# Autodesk Inventor assembly: 810004_X0X
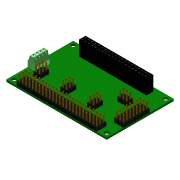
[picture p0: Inventor's stored thumbnail of the model, 180x180]
Saved by Autodesk Inventor 2015 (Build 190159000, 159)
## iProperties
Created: 2014-08-28
Part Number: 810004_X0X
Document SubType Name: Assembly
Designer: david
Author: david
## Documents named in this file (3)
- C:\SharedDrive\Dropbox\FAST Robotics\Products\818004_Power Shield\MECH\810004_Power Shield\810004A\810004A_X0X.iam
- C:\SharedDrive\Dropbox\FAST Robotics\Products\818004_Power Shield\MECH\810004_Power Shield\810004A\810004A_XXX.iam
- C:\SharedDrive\Dropbox\FAST Robotics\Library\784001_CONN HEADER .1in SINGLE STR 40POS\CONN HEADER .1in SINGLE STR 40POS.ipt
## Components (97 placed, 2 different names)
1. 810004A_XXX:1 [sub-assembly] — Flush:1, Flush:2, Flush:3, Mate:1, Mate:2, Mate:3, Mate:4, Flush:4, Flush:5, Flush:6, Flush:7, Flush:8, Flush:10, Flush:11
2. CONN HEADER .1in SINGLE STR 40POS:1
3. CONN HEADER .1in SINGLE STR 40POS:2
4. CONN HEADER .1in SINGLE STR 40POS:3 — Mate:1, Flush:4, Flush:8
5. CONN HEADER .1in SINGLE STR 40POS:4
6. CONN HEADER .1in SINGLE STR 40POS:5
7. CONN HEADER .1in SINGLE STR 40POS:6
8. CONN HEADER .1in SINGLE STR 40POS:7
9. CONN HEADER .1in SINGLE STR 40POS:8
10. CONN HEADER .1in SINGLE STR 40POS:9
11. CONN HEADER .1in SINGLE STR 40POS:10
12. CONN HEADER .1in SINGLE STR 40POS:11
13. CONN HEADER .1in SINGLE STR 40POS:12
14. CONN HEADER .1in SINGLE STR 40POS:13
15. CONN HEADER .1in SINGLE STR 40POS:14
16. CONN HEADER .1in SINGLE STR 40POS:15
17. CONN HEADER .1in SINGLE STR 40POS:16
18. CONN HEADER .1in SINGLE STR 40POS:17
19. CONN HEADER .1in SINGLE STR 40POS:18
20. CONN HEADER .1in SINGLE STR 40POS:19
21. CONN HEADER .1in SINGLE STR 40POS:20
22. CONN HEADER .1in SINGLE STR 40POS:21
23. CONN HEADER .1in SINGLE STR 40POS:22
24. CONN HEADER .1in SINGLE STR 40POS:23
25. CONN HEADER .1in SINGLE STR 40POS:24 — Mate:5
26. CONN HEADER .1in SINGLE STR 40POS:25
27. CONN HEADER .1in SINGLE STR 40POS:28
28. CONN HEADER .1in SINGLE STR 40POS:29
29. CONN HEADER .1in SINGLE STR 40POS:30
30. CONN HEADER .1in SINGLE STR 40POS:31
31. CONN HEADER .1in SINGLE STR 40POS:32
32. CONN HEADER .1in SINGLE STR 40POS:33
33. CONN HEADER .1in SINGLE STR 40POS:34
34. CONN HEADER .1in SINGLE STR 40POS:35
35. CONN HEADER .1in SINGLE STR 40POS:36
36. CONN HEADER .1in SINGLE STR 40POS:37
37. CONN HEADER .1in SINGLE STR 40POS:38
38. CONN HEADER .1in SINGLE STR 40POS:39
39. CONN HEADER .1in SINGLE STR 40POS:40
40. CONN HEADER .1in SINGLE STR 40POS:41
41. CONN HEADER .1in SINGLE STR 40POS:42
42. CONN HEADER .1in SINGLE STR 40POS:43 — Mate:5
43. CONN HEADER .1in SINGLE STR 40POS:44
44. CONN HEADER .1in SINGLE STR 40POS:45
45. CONN HEADER .1in SINGLE STR 40POS:46
46. CONN HEADER .1in SINGLE STR 40POS:47 — Mate:2
47. CONN HEADER .1in SINGLE STR 40POS:48
48. CONN HEADER .1in SINGLE STR 40POS:49
49. CONN HEADER .1in SINGLE STR 40POS:50 — Flush:5
50. CONN HEADER .1in SINGLE STR 40POS:27
51. CONN HEADER .1in SINGLE STR 40POS:51
52. CONN HEADER .1in SINGLE STR 40POS:52
53. CONN HEADER .1in SINGLE STR 40POS:53
54. CONN HEADER .1in SINGLE STR 40POS:54
55. CONN HEADER .1in SINGLE STR 40POS:55
56. CONN HEADER .1in SINGLE STR 40POS:56
57. CONN HEADER .1in SINGLE STR 40POS:57 — Mate:4
58. CONN HEADER .1in SINGLE STR 40POS:58
59. CONN HEADER .1in SINGLE STR 40POS:59
60. CONN HEADER .1in SINGLE STR 40POS:60
61. CONN HEADER .1in SINGLE STR 40POS:61
62. CONN HEADER .1in SINGLE STR 40POS:62
63. CONN HEADER .1in SINGLE STR 40POS:63
64. CONN HEADER .1in SINGLE STR 40POS:64
65. CONN HEADER .1in SINGLE STR 40POS:65 — Flush:10
66. CONN HEADER .1in SINGLE STR 40POS:66
67. CONN HEADER .1in SINGLE STR 40POS:67
68. CONN HEADER .1in SINGLE STR 40POS:68
69. CONN HEADER .1in SINGLE STR 40POS:69
70. CONN HEADER .1in SINGLE STR 40POS:70
71. CONN HEADER .1in SINGLE STR 40POS:71
72. CONN HEADER .1in SINGLE STR 40POS:72 — Flush:7
73. CONN HEADER .1in SINGLE STR 40POS:73
74. CONN HEADER .1in SINGLE STR 40POS:26
75. CONN HEADER .1in SINGLE STR 40POS:74
76. CONN HEADER .1in SINGLE STR 40POS:75
77. CONN HEADER .1in SINGLE STR 40POS:76
78. CONN HEADER .1in SINGLE STR 40POS:77
79. CONN HEADER .1in SINGLE STR 40POS:78
80. CONN HEADER .1in SINGLE STR 40POS:79
81. CONN HEADER .1in SINGLE STR 40POS:80
82. CONN HEADER .1in SINGLE STR 40POS:81
83. CONN HEADER .1in SINGLE STR 40POS:82
84. CONN HEADER .1in SINGLE STR 40POS:83
85. CONN HEADER .1in SINGLE STR 40POS:84
86. CONN HEADER .1in SINGLE STR 40POS:85
87. CONN HEADER .1in SINGLE STR 40POS:86
88. CONN HEADER .1in SINGLE STR 40POS:87
89. CONN HEADER .1in SINGLE STR 40POS:88
90. CONN HEADER .1in SINGLE STR 40POS:89 — Flush:11
91. CONN HEADER .1in SINGLE STR 40POS:90
92. CONN HEADER .1in SINGLE STR 40POS:91
93. CONN HEADER .1in SINGLE STR 40POS:92
94. CONN HEADER .1in SINGLE STR 40POS:93
95. CONN HEADER .1in SINGLE STR 40POS:94
96. CONN HEADER .1in SINGLE STR 40POS:95
97. CONN HEADER .1in SINGLE STR 40POS:96 — Mate:3, Flush:6
## Component patterns: GPIOAx8 (24 elements), GPIOBx8 (24 elements), GPIOCx8 (24 elements), GPIODx8 (24 elements)
## Relationships (15: Flush 10, Mate 5)
- Flush:1: 810004A_XXX:1
- Flush:2: 810004A_XXX:1
- Flush:3: 810004A_XXX:1
- Mate:1: 810004A_XXX:1 ↔ CONN HEADER .1in SINGLE STR 40POS:3
- Mate:2: 810004A_XXX:1 ↔ CONN HEADER .1in SINGLE STR 40POS:47
- Mate:3: 810004A_XXX:1 ↔ CONN HEADER .1in SINGLE STR 40POS:96
- Mate:4: 810004A_XXX:1 ↔ CONN HEADER .1in SINGLE STR 40POS:57
- Flush:4: 810004A_XXX:1 ↔ CONN HEADER .1in SINGLE STR 40POS:3
- Flush:5: 810004A_XXX:1 ↔ CONN HEADER .1in SINGLE STR 40POS:50
- Flush:6: 810004A_XXX:1 ↔ CONN HEADER .1in SINGLE STR 40POS:96
- Flush:7: 810004A_XXX:1 ↔ CONN HEADER .1in SINGLE STR 40POS:72
- Flush:8 (7.62 mm): 810004A_XXX:1 ↔ CONN HEADER .1in SINGLE STR 40POS:3
- Flush:10 (7.62 mm): 810004A_XXX:1 ↔ CONN HEADER .1in SINGLE STR 40POS:65
- Flush:11 (-12.7 mm): 810004A_XXX:1 ↔ CONN HEADER .1in SINGLE STR 40POS:89
- Mate:5 (0.127 mm): CONN HEADER .1in SINGLE STR 40POS:24 ↔ CONN HEADER .1in SINGLE STR 40POS:43
